# Autodesk Inventor assembly: BaseLinkSide
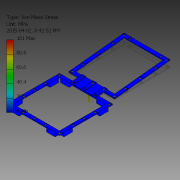
[picture p0: Inventor's stored thumbnail of the model, 180x180]
Saved by Autodesk Inventor 2014 SP1 (Build 180222100, 222)
## iProperties
Created: 2015-04-03
Part Number: BaseLinkSide
Document SubType Name: Assembly
Designer: Erin
Author: Erin
## Documents named in this file (10)
- C:\Users\Erin\Desktop\RDAS Base\BaseLinkSide.iam
- C:\Users\Erin\Desktop\RDAS Base\Side.ipt
- C:\Users\Erin\Desktop\RDAS Base\SideLink.ipt
- C:\Users\Erin\Desktop\RDAS Base\Base.ipt
- C:\Users\Erin\Desktop\RDAS Base\BaseLinkSide\AIP\FEA\bdkw11n5s.fins
- C:\Users\Erin\Desktop\RDAS Base\BaseLinkSide\AIP\FEA\bdkw11n6o.fsat
- C:\Users\Erin\Desktop\RDAS Base\BaseLinkSide\AIP\FEA\bdkw11n6o.ftes
- C:\Users\Erin\Desktop\RDAS Base\BaseLinkSide\AIP\FEA\bdkw11n6o.fwiz
- C:\Users\Erin\Desktop\RDAS Base\BaseLinkSide\AIP\FEA\bdkw11n9c.fmsh
- C:\Users\Erin\Desktop\RDAS Base\BaseLinkSide\AIP\FEA\bdkw11n9d.fres
## Components (3 placed, 3 different names)
1. Side:1 — Insert:1, Insert:2
2. SideLink:1 — Insert:1, Insert:2, Insert:3, Insert:4
3. Base:1 — Insert:3, Insert:4
## Relationships (4: Insert 4)
- Insert:1: Side:1 ↔ SideLink:1
- Insert:2: Side:1 ↔ SideLink:1
- Insert:3: SideLink:1 ↔ Base:1
- Insert:4: SideLink:1 ↔ Base:1
## Named parameters: sa_0 = 0, sa_1 = -0, sa_2 = 5500
note: some values were not read from the file. Shown as the stored number, unit unknown: "sa_0", "sa_1", "sa_2".
